# Autodesk Inventor assembly: Press_Assembly
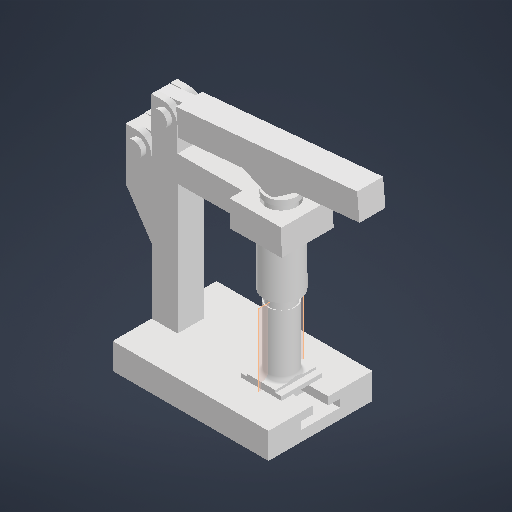
[picture p0: Inventor's stored thumbnail of the model, 512x512]
Saved by Autodesk Inventor 2026.1 (Build 301233020, 233B)
## iProperties
Created: 2025-09-29
Part Number: Press_Assembly
Document SubType Name: Assembly
Designer: Gamec
Author: Gamec
## Documents named in this file (8)
- C:\Users\Gamec\OneDrive\Desktop\USCRC\Projects\AcidBaseRockets\Press\Press_Assembly.iam
- C:\Users\Gamec\OneDrive\Desktop\USCRC\Projects\AcidBaseRockets\Press\Press_Base.ipt
- C:\Users\Gamec\OneDrive\Desktop\USCRC\Projects\AcidBaseRockets\Press\Press_Lower_Arm.ipt
- C:\Users\Gamec\OneDrive\Desktop\USCRC\Projects\AcidBaseRockets\Press\Press_Head.ipt
- C:\Users\Gamec\OneDrive\Desktop\USCRC\Projects\AcidBaseRockets\Press\Press_Mandrel.ipt
- C:\Users\Gamec\OneDrive\Desktop\USCRC\Projects\AcidBaseRockets\DRAFTS\MOULD.ipt
- C:\Users\Gamec\OneDrive\Desktop\USCRC\Projects\AcidBaseRockets\Press\Press_Upper_Arm.ipt
- C:\Users\Gamec\OneDrive\Desktop\USCRC\Projects\AcidBaseRockets\Press\Pin.ipt
## Components (8 placed, 7 different names)
1. Press_Base:1 — Rotational:1, Mate:1, Mate:2, Mate:3, Rotational:3
2. Press_Lower_Arm:1 — Rotational:1, Cylindrical:1, Rotational:2, Rotational:4
3. Press_Head:1 — Cylindrical:1
4. Press_Mandrel:1 — Mate:1, Mate:2, Mate:3, Mate:4
5. MOULD:1 — Mate:4
6. Press_Upper_Arm:1 — Rotational:2
7. Pin:1 — Rotational:3
8. Pin:2 — Rotational:4
## Relationships (9: RevoluteJoint 4, Mate 4, CylindricalJoint 1)
- Rotational:1 [RevoluteJoint] (0.0635 mm): Press_Base:1 ↔ Press_Lower_Arm:1
- Cylindrical:1: Press_Lower_Arm:1 ↔ Press_Head:1
- Mate:1: Press_Base:1 ↔ Press_Mandrel:1
- Mate:2: Press_Base:1 ↔ Press_Mandrel:1
- Mate:3 (0.127 mm): Press_Base:1 ↔ Press_Mandrel:1
- Mate:4: Press_Mandrel:1 ↔ MOULD:1
- Rotational:2 [RevoluteJoint]: Press_Lower_Arm:1 ↔ Press_Upper_Arm:1
- Rotational:3 [RevoluteJoint]: Press_Base:1 ↔ Pin:1
- Rotational:4 [RevoluteJoint]: Press_Lower_Arm:1 ↔ Pin:2
